# Autodesk Inventor assembly: TopRoller-ver1-1111-2019
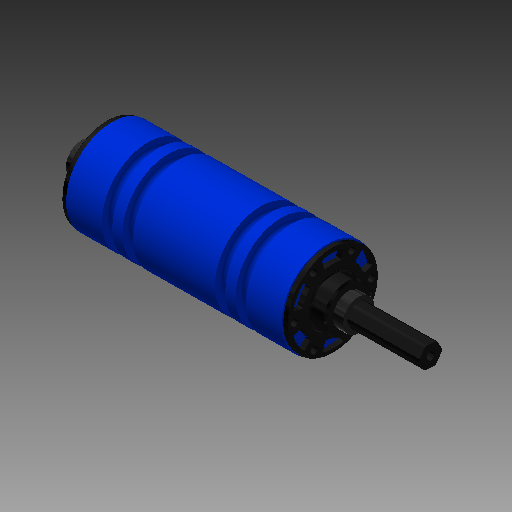
[picture p0: Inventor's stored thumbnail of the model, 512x512]
Saved by Autodesk Inventor 2018 (Build 220112000, 112)
## iProperties
Created: 2020-01-25
Part Number: TopRoller-ver1-1111-2019
Document SubType Name: Assembly
Designer: JMHal
Author: JMHal
## Documents named in this file (5)
- F:\GrabCad\2020 Infinite Recharge\Storage\Assemblies\TopRoller-ver1-1111-2019.iam
- F:\GrabCad\Resources\VEXpro Resources\Versa Motion\VersaHub(0.5inHex)-1111-2016.ipt
- F:\GrabCad\2020 Infinite Recharge\Storage\Parts\Roller-ver3-1111-2019.ipt
- F:\GrabCad\Resources\VEXpro Resources\Shafts\0.5inThunderHexShaft(8in(modified))-1111-2016.ipt
- F:\GrabCad\Resources\VEXpro Resources\Spacers\0.25inAcetalSpacer(0.5inHex)-1111-2016.ipt
## Components (6 placed, 4 different names)
1. VersaHub(0.5inHex)-1111-2016:1 — Mate:12, Mate:13, Cylindrical:2, Mate:14
2. Roller-ver3-1111-2019:1 — Mate:10, Mate:11, Mate:12, Mate:13, Mate:16
3. VersaHub(0.5inHex)-1111-2016:2 — Mate:10, Mate:11, Mate:15, Mate:16, Mate:17
4. 0.5inThunderHexShaft(8in(modified))-1111-2016:1 — Cylindrical:1, Cylindrical:2, Flush:1
5. 0.25inAcetalSpacer(0.5inHex)-1111-2016:1 — Mate:15, Mate:17
6. 0.25inAcetalSpacer(0.5inHex)-1111-2016:2 — Cylindrical:1, Mate:14, Flush:1
## Relationships (11: Mate 8, CylindricalJoint 2, Flush 1)
- Mate:10: Roller-ver3-1111-2019:1 ↔ VersaHub(0.5inHex)-1111-2016:2
- Mate:11: Roller-ver3-1111-2019:1 ↔ VersaHub(0.5inHex)-1111-2016:2
- Mate:12: VersaHub(0.5inHex)-1111-2016:1 ↔ Roller-ver3-1111-2019:1
- Mate:13: VersaHub(0.5inHex)-1111-2016:1 ↔ Roller-ver3-1111-2019:1
- Cylindrical:1: 0.5inThunderHexShaft(8in(modified))-1111-2016:1 ↔ 0.25inAcetalSpacer(0.5inHex)-1111-2016:2
- Cylindrical:2: VersaHub(0.5inHex)-1111-2016:1 ↔ 0.5inThunderHexShaft(8in(modified))-1111-2016:1
- Mate:14: VersaHub(0.5inHex)-1111-2016:1 ↔ 0.25inAcetalSpacer(0.5inHex)-1111-2016:2
- Mate:15: VersaHub(0.5inHex)-1111-2016:2 ↔ 0.25inAcetalSpacer(0.5inHex)-1111-2016:1
- Mate:16: Roller-ver3-1111-2019:1 ↔ VersaHub(0.5inHex)-1111-2016:2
- Mate:17: VersaHub(0.5inHex)-1111-2016:2 ↔ 0.25inAcetalSpacer(0.5inHex)-1111-2016:1
- Flush:1 (63.5 mm): 0.5inThunderHexShaft(8in(modified))-1111-2016:1 ↔ 0.25inAcetalSpacer(0.5inHex)-1111-2016:2
